# Autodesk Inventor assembly: tail_p1
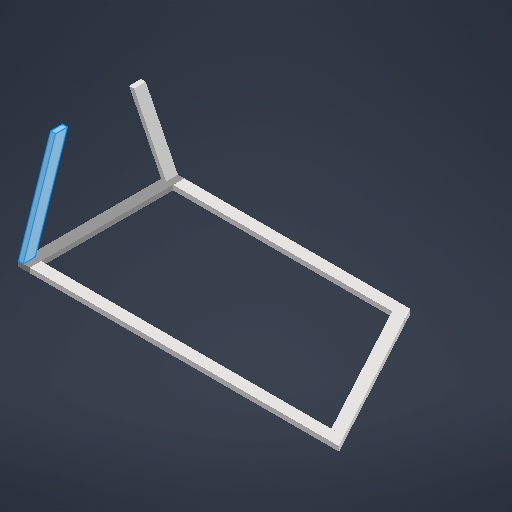
[picture p0: Inventor's stored thumbnail of the model, 512x512]
Saved by Autodesk Inventor 2027.1 (Build 311270010, 270A)
## iProperties
Created: 2026-09-01
Part Number: tail_p1
Document SubType Name: Assembly
Designer: jorda
Author: jorda
## Documents named in this file (6)
- C:\Users\jorda\OneDrive\Documents\GitHub\USC-ASME-TigerBurn-2026\CAD\Tail\tail_p1.iam
- C:\Users\jorda\OneDrive\Documents\GitHub\USC-ASME-TigerBurn-2026\CAD\Tail\2x4x48.ipt
- C:\Users\jorda\OneDrive\Documents\GitHub\USC-ASME-TigerBurn-2026\CAD\Tail\S_2x4x50.56.ipt
- C:\Users\jorda\OneDrive\Documents\GitHub\USC-ASME-TigerBurn-2026\CAD\Tail\S_2x4x72.ipt
- C:\Users\jorda\OneDrive\Documents\GitHub\USC-ASME-TigerBurn-2026\CAD\Tail\S_2x4x96.ipt
- C:\Users\jorda\OneDrive\Documents\GitHub\USC-ASME-TigerBurn-2026\CAD\Tail\S_2x4x39.27.ipt
## Components (6 placed, 5 different names)
1. 2x4x48:1 — Mate:3, Flush:5, Flush:6, Mate:4, Flush:7, Flush:8, Mate:6, Mate:7, Flush:9, Mate:8, Flush:10
2. S_2x4x50.56:1
3. S_2x4x72:1 — Mate:3, Flush:5, Flush:6
4. S_2x4x96:1 — Mate:4, Flush:7, Flush:8
5. S_2x4x39.27:1 — Mate:6, Mate:7, Flush:9
6. S_2x4x39.27:2 — Mate:8, Flush:10
## Relationships (11: Flush 6, Mate 5)
- Mate:3: 2x4x48:1 ↔ S_2x4x72:1
- Flush:5: 2x4x48:1 ↔ S_2x4x72:1
- Flush:6: 2x4x48:1 ↔ S_2x4x72:1
- Mate:4: 2x4x48:1 ↔ S_2x4x96:1
- Flush:7: 2x4x48:1 ↔ S_2x4x96:1
- Flush:8: 2x4x48:1 ↔ S_2x4x96:1
- Mate:6: 2x4x48:1 ↔ S_2x4x39.27:1
- Mate:7: 2x4x48:1 ↔ S_2x4x39.27:1
- Flush:9: 2x4x48:1 ↔ S_2x4x39.27:1
- Mate:8: 2x4x48:1 ↔ S_2x4x39.27:2
- Flush:10: 2x4x48:1 ↔ S_2x4x39.27:2
